# Autodesk Inventor assembly: PortaPiezas
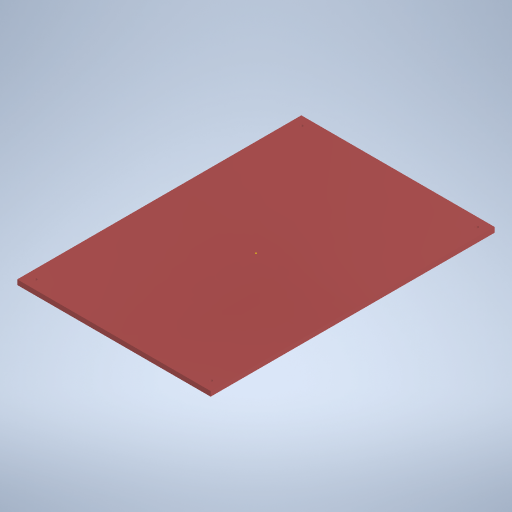
[picture p0: Inventor's stored thumbnail of the model, 512x512]
Saved by Autodesk Inventor 2023.1 (Build 271208000, 208)
## iProperties
Created: 2022-11-11
Part Number: PortaPiezas
Document SubType Name: Assembly
Designer: Daniel Peña
Author: Daniel Peña
## Documents named in this file (3)
- C:\Users\danie\Documents\UN\ProyectoRobotica\CAD\V3 - BigChungus\PortaPiezas.iam
- C:\Users\danie\Documents\UN\ProyectoRobotica\CAD\V3 - BigChungus\Base.ipt
- C:\Users\danie\Documents\UN\ProyectoRobotica\CAD\V3 - BigChungus\PortaPiezas.ipt
## Components (2 placed, 2 different names)
1. Base:1 — Insert:1, Insert:2, Insert:3, Insert:4
2. PortaPiezas:1 — Insert:1, Insert:2, Insert:3, Insert:4
## Relationships (4: Insert 4)
- Insert:1: Base:1 ↔ PortaPiezas:1
- Insert:2: Base:1 ↔ PortaPiezas:1
- Insert:3: Base:1 ↔ PortaPiezas:1
- Insert:4: Base:1 ↔ PortaPiezas:1
